# Autodesk Inventor assembly: Vehicle Registration Plate Final
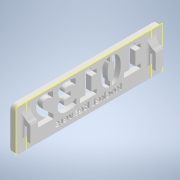
[picture p0: Inventor's stored thumbnail of the model, 180x180]
Saved by Autodesk Inventor 2020 (Build 240168000, 168)
## iProperties
Created: 2020-01-20
Part Number: Vehicle Registration Plate Final
Document SubType Name: Assembly
Designer: maple
Author: maple
## Documents named in this file (2)
- C:\Users\maple\Documents\GitHub\3D-Models\Robotics\Vehicle Registration Plate Final.iam
- C:\Users\maple\Documents\GitHub\3D-Models\Robotics\Vehicle Registration Plate Final.ipt
## Components (1 placed, 1 different names)
1. Vehicle Registration Plate Final:1 — Mate:1, Mate:2
## Relationships (2: Mate 2)
- Mate:1: Vehicle Registration Plate Final:1
- Mate:2: Vehicle Registration Plate Final:1
